# Autodesk Inventor assembly: EnsambleCajaElectrica
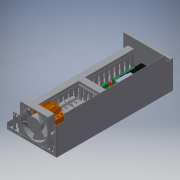
[picture p0: Inventor's stored thumbnail of the model, 180x180]
Saved by Autodesk Inventor 2017 (Build 210142000, 142)
## iProperties
Created: 2020-11-13
Part Number: EnsambleCajaElectrica
Document SubType Name: Assembly
Designer: USUARIO
Author: USUARIO
## Documents named in this file (10)
- D:\Laboratorio\Autoclave\Autoclave Horizontal\Sin Precamara\2019\Autoclave 40L con Vacio Angelica Castañeda #004588041 OP2019149\Modelo 3D\EnsambleCajaElectrica.iam
- D:\Laboratorio\Autoclave\Autoclave Horizontal\Sin Precamara\2019\Autoclave 40L con Vacio Angelica Castañeda #004588041 OP2019149\Modelo 3D\NextionControlV3.iam
- C:\Users\USUARIO\Documents\Inventor\Canaleta 30x60 450mm.iam
- C:\Users\USUARIO\Documents\Inventor\Canaleta 30x60 120mm.iam
- C:\Modelos 3D y DXF\Ex9C 25-38-NOARK.stp\Ex9C 25-38-NOARK.ipt
- C:\Modelos 3D y DXF\B1A-NOARK.stp\75856.ipt
- C:\Modelos 3D y DXF\B1A-NOARK.stp\B1A-NOARK.ipt
- C:\Modelos 3D y DXF\SSR\a24125pg.ipt
- D:\Laboratorio\Autoclave\Autoclave Horizontal\Sin Precamara\2019\Autoclave 40L con Vacio Angelica Castañeda #004588041 OP2019149\Modelo 3D\CAJA CONEXIONES ACH-40L-2019 MOD2020.ipt
- D:\Laboratorio\Autoclave\Autoclave Horizontal\Sin Precamara\2019\Autoclave 40L con Vacio Angelica Castañeda #004588041 OP2019149\Modelo 3D\VENTILADOR 11X11.ipt
## Components (12 placed, 9 different names)
1. NextionControlV3:1 [sub-assembly] — Mate:30, Mate:31
2. Canaleta 30x60 450mm:1 [sub-assembly] — Mate:9, Mate:14, Mate:22, Mate:23, Mate:25, Mate:35, Mate:36
3. Canaleta 30x60 120mm:1 [sub-assembly] — Mate:9, Mate:12, Mate:28
4. Canaleta 30x60 450mm:2 [sub-assembly] — Mate:12, Mate:26, Mate:27
5. Ex9C 25-38-NOARK:1 — Mate:14, Mate:29
6. B1A-NOARK:1 — Mate:22, Mate:32
7. CAJA CONEXIONES ACH-40L-2019 MOD2020:1 — Mate:23, Mate:25, Mate:26, Mate:27, Mate:28, Mate:29, Mate:30, Mate:31, Mate:32, Mate:33, Mate:34, Mate:37, Mate:38, Mate:39, Mate:40
8. 75856:1 — Mate:33, Mate:35
9. 75856:2 — Mate:34, Mate:36
10. a24125pg:1 — Mate:39
11. VENTILADOR 11X11:1 — Mate:37, Mate:38
12. a24125pg:2 — Mate:40
## Relationships (21: Mate 21)
- Mate:9: Canaleta 30x60 450mm:1 ↔ Canaleta 30x60 120mm:1
- Mate:12: Canaleta 30x60 120mm:1 ↔ Canaleta 30x60 450mm:2
- Mate:14 (95 mm): Canaleta 30x60 450mm:1 ↔ Ex9C 25-38-NOARK:1
- Mate:22 (10 mm): Canaleta 30x60 450mm:1 ↔ B1A-NOARK:1
- Mate:23: Canaleta 30x60 450mm:1 ↔ CAJA CONEXIONES ACH-40L-2019 MOD2020:1
- Mate:25: Canaleta 30x60 450mm:1 ↔ CAJA CONEXIONES ACH-40L-2019 MOD2020:1
- Mate:26: Canaleta 30x60 450mm:2 ↔ CAJA CONEXIONES ACH-40L-2019 MOD2020:1
- Mate:27: Canaleta 30x60 450mm:2 ↔ CAJA CONEXIONES ACH-40L-2019 MOD2020:1
- Mate:28: Canaleta 30x60 120mm:1 ↔ CAJA CONEXIONES ACH-40L-2019 MOD2020:1
- Mate:29 (-2 mm): Ex9C 25-38-NOARK:1 ↔ CAJA CONEXIONES ACH-40L-2019 MOD2020:1
- Mate:30 (15 mm): NextionControlV3:1 ↔ CAJA CONEXIONES ACH-40L-2019 MOD2020:1
- Mate:31 (10 mm): NextionControlV3:1 ↔ CAJA CONEXIONES ACH-40L-2019 MOD2020:1
- Mate:32 (2 mm): B1A-NOARK:1 ↔ CAJA CONEXIONES ACH-40L-2019 MOD2020:1
- Mate:33: CAJA CONEXIONES ACH-40L-2019 MOD2020:1 ↔ 75856:1
- Mate:34: CAJA CONEXIONES ACH-40L-2019 MOD2020:1 ↔ 75856:2
- Mate:35 (22 mm): Canaleta 30x60 450mm:1 ↔ 75856:1
- Mate:36 (22 mm): Canaleta 30x60 450mm:1 ↔ 75856:2
- Mate:37: CAJA CONEXIONES ACH-40L-2019 MOD2020:1 ↔ VENTILADOR 11X11:1
- Mate:38 (10 mm): CAJA CONEXIONES ACH-40L-2019 MOD2020:1 ↔ VENTILADOR 11X11:1
- Mate:39: CAJA CONEXIONES ACH-40L-2019 MOD2020:1 ↔ a24125pg:1
- Mate:40: CAJA CONEXIONES ACH-40L-2019 MOD2020:1 ↔ a24125pg:2
